# Autodesk Inventor assembly: 偏心軸ユニット
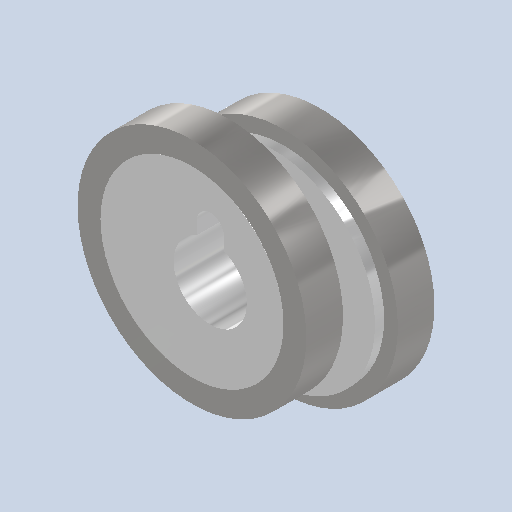
[picture p0: Inventor's stored thumbnail of the model, 512x512]
Saved by Autodesk Inventor 2024 (Build 280153000, 153)
## iProperties
Created: 2023-05-29
Part Number: 偏心軸ユニット
Document SubType Name: Assembly
Designer: yuta2
Author: yuta2
## Documents named in this file (3)
- C:\Users\yuta2\Documents\Inventor\CycloidDrive\サイクロイド減速機_大型\偏心軸ユニット.iam
- C:\Users\yuta2\Documents\Inventor\CycloidDrive\サイクロイド減速機_大型\偏心軸板.ipt
- C:\Users\yuta2\Documents\Inventor\CycloidDrive\ベアリング\ベアリングDDA-2520.ipt
## Components (4 placed, 2 different names)
1. 偏心軸板:1 — 回転:1, リジッド:1, 回転:3
2. 偏心軸板:2 — 回転:1, リジッド:1, 回転:2
3. ベアリングDDA-2520:1 — 回転:3
4. ベアリングDDA-2520:2 — 回転:2
## Relationships (4: RevoluteJoint 3, WeldJoint 1)
- 回転:1 [RevoluteJoint]: 偏心軸板:1 ↔ 偏心軸板:2
- リジッド:1 [WeldJoint]: 偏心軸板:1 ↔ 偏心軸板:2
- 回転:2 [RevoluteJoint]: 偏心軸板:2 ↔ ベアリングDDA-2520:2
- 回転:3 [RevoluteJoint]: 偏心軸板:1 ↔ ベアリングDDA-2520:1
